# Autodesk Inventor assembly: Radial Engine Assembly_Jen
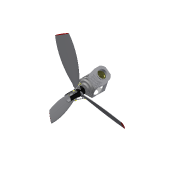
[picture p0: Inventor's stored thumbnail of the model, 180x180]
Saved by Autodesk Inventor 2022 Beta2 (Build 260130000, 130) ContinuousBuild 0
## iProperties
Created: 2013-03-12
Part Number: Radial Engine Assembly_Jen
Document SubType Name: Assembly
Designer: jmacmillan
Author: jmacmillan
## Documents named in this file (11)
- C:\Autodesk Inventor 2021 Intro Practice Files\Engine\Radial Engine Final.iam
- C:\Autodesk Inventor 2021 Intro Practice Files\Engine\RBlock.ipt
- C:\Autodesk Inventor 2021 Intro Practice Files\Engine\Rcylinder.ipt
- C:\Autodesk Inventor 2021 Intro Practice Files\Engine\Crankshaft.ipt
- C:\Autodesk Inventor 2021 Intro Practice Files\Engine\Master Rod1.ipt
- C:\Autodesk Inventor 2021 Intro Practice Files\Engine\Piston head pin.ipt
- C:\Autodesk Inventor 2021 Intro Practice Files\Engine\Piston head.ipt
- C:\Autodesk Inventor 2021 Intro Practice Files\Engine\Hub.ipt
- C:\Autodesk Inventor 2021 Intro Practice Files\Engine\Shuttle.ipt
- C:\Autodesk Inventor 2021 Intro Practice Files\Engine\Pro_blade.ipt
- C:\Autodesk Inventor 2021 Intro Practice Files\Engine\Prop_Conrod.ipt
## Components (14 placed, 10 different names)
1. RBlock:1 — Rigid:1, Cylindrical:2
2. Rcylinder:1 — Rigid:1, Cylindrical:1
3. Crankshaft:1 — Rotational:1, Cylindrical:2, Rigid:3
4. Master Rod1:1 — Rotational:1, Rotational:2
5. Piston head pin:1 — Rigid:2, Rotational:2
6. Piston head:1 — Rigid:2, Cylindrical:1
7. Hub:1 — Rigid:3, Cylindrical:3, Angle:1, Rotational:3, Rotational:4, Rotational:5
8. Shuttle:1 — Cylindrical:3, Angle:1, Ball:2, Ball:5, Ball:6
9. Pro_blade:1 — Rotational:3, Ball:1
10. Prop_Conrod:1 — Ball:1, Ball:2
11. Pro_blade:2 — Rotational:4
12. Prop_Conrod:2 — Ball:5
13. Pro_blade:3 — Rotational:5
14. Prop_Conrod:3 — Ball:6
## Relationships (18: BallJoint 6, RevoluteJoint 5, WeldJoint 3, CylindricalJoint 3, Angle 1)
- Rigid:1 [WeldJoint]: RBlock:1 ↔ Rcylinder:1
- Rotational:1 [RevoluteJoint] (-27.94 mm): Crankshaft:1 ↔ Master Rod1:1
- Rigid:2 [WeldJoint] (-1.27 mm): Piston head pin:1 ↔ Piston head:1
- Rotational:2 [RevoluteJoint]: Master Rod1:1 ↔ Piston head pin:1
- Cylindrical:1: Rcylinder:1 ↔ Piston head:1
- Cylindrical:2: RBlock:1 ↔ Crankshaft:1
- Rigid:3 [WeldJoint]: Crankshaft:1 ↔ Hub:1
- Cylindrical:3: Hub:1 ↔ Shuttle:1
- Angle:1 (180 deg): Hub:1 ↔ Shuttle:1
- Rotational:3 [RevoluteJoint]: Hub:1 ↔ Pro_blade:1
- Ball:1: Pro_blade:1 ↔ Prop_Conrod:1
- Ball:2: Shuttle:1 ↔ Prop_Conrod:1
- [BallJoint]: Pro_blade:2 ↔ Prop_Conrod:2
- [BallJoint]: Pro_blade:3 ↔ Prop_Conrod:3
- Rotational:4 [RevoluteJoint]: Hub:1 ↔ Pro_blade:2
- Ball:5: Shuttle:1 ↔ Prop_Conrod:2
- Rotational:5 [RevoluteJoint]: Hub:1 ↔ Pro_blade:3
- Ball:6: Shuttle:1 ↔ Prop_Conrod:3
